# Autodesk Inventor assembly: Energy Chain Tensioner piece
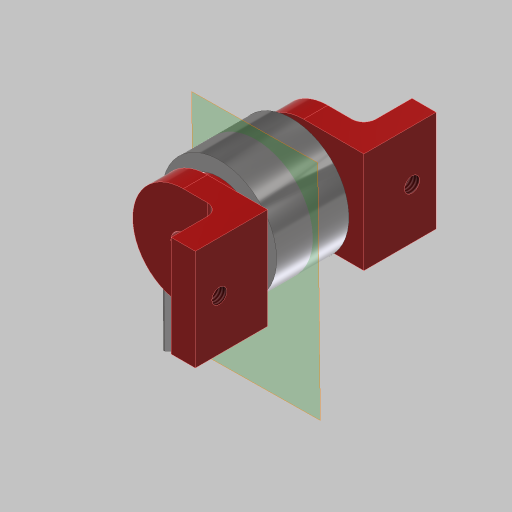
[picture p0: Inventor's stored thumbnail of the model, 512x512]
Saved by Autodesk Inventor 2023.5 (Build 275446000, 446)
## iProperties
Created: 2025-01-21
Part Number: Energy Chain Tensioner piece
Document SubType Name: Assembly
Designer: slick
Author: slick
## Documents named in this file (4)
- C:\Users\slick\OneDrive\Desktop\2025-ReefScape---CAD\Elevator\EL2\Energy Chain Tensioner piece.iam
- C:\Users\slick\OneDrive\Desktop\2025-ReefScape---CAD\COMMON PARTS\BEARINGS\Ball Bearing 1_4x11_16x5_16 Sealed 1602DC 1602-2RS.ipt
- C:\Users\slick\OneDrive\Desktop\2025-ReefScape---CAD\COMMON PARTS\9293K560_STAINLESS STEEL CONSTANT-FORCE SPRING.ipt
- C:\Users\slick\OneDrive\Desktop\2025-ReefScape---CAD\Elevator\EL2\EL2-031.ipt
## Components (5 placed, 3 different names)
1. EL2-031:1 — Mate:1, Flush:1, Mate:3, Mate:4, Mate:5, Flush:3
2. Ball Bearing 1_4x11_16x5_16 Sealed 1602DC 1602-2RS:1 — Mate:1, Flush:1
3. EL2-031:2 — Mate:3, Mate:4, Mate:6, Flush:3
4. Ball Bearing 1_4x11_16x5_16 Sealed 1602DC 1602-2RS:2
5. 9293K560_STAINLESS STEEL CONSTANT-FORCE SPRING:1 — Mate:5, Mate:6
## Relationships (9: Mate 6, Flush 3)
- Mate:1: EL2-031:1 ↔ Ball Bearing 1_4x11_16x5_16 Sealed 1602DC 1602-2RS:1
- Flush:1 (3.175 mm): EL2-031:1 ↔ Ball Bearing 1_4x11_16x5_16 Sealed 1602DC 1602-2RS:1
- [Mate]: EL2-031:2 ↔ Ball Bearing 1_4x11_16x5_16 Sealed 1602DC 1602-2RS:2
- [Flush] (3.175 mm): EL2-031:2 ↔ Ball Bearing 1_4x11_16x5_16 Sealed 1602DC 1602-2RS:2
- Mate:3: EL2-031:1 ↔ EL2-031:2
- Mate:4: EL2-031:1 ↔ EL2-031:2
- Mate:5: EL2-031:1 ↔ 9293K560_STAINLESS STEEL CONSTANT-FORCE SPRING:1
- Mate:6 (3.175 mm): EL2-031:2 ↔ 9293K560_STAINLESS STEEL CONSTANT-FORCE SPRING:1
- Flush:3: EL2-031:1 ↔ EL2-031:2
## Named parameters: d2_d0 = 0 mm, d3_d1 = 3.175 mm
